# Autodesk Inventor assembly: blue wheel
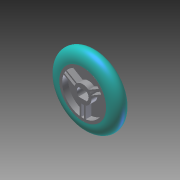
[picture p0: Inventor's stored thumbnail of the model, 180x180]
Saved by Autodesk Inventor 2012 (Build 160160000, 160)
## iProperties
Created: 2013-10-11
Part Number: blue wheel
Document SubType Name: Assembly
Designer: Bryce
Author: Bryce
## Documents named in this file (3)
- C:\Users\Bryce\Dropbox\Inventor Design Project Files\Independent Swerves\Inventor 2012\blue wheel.iam
- C:\Users\Bryce\Dropbox\Inventor Design Project Files\Independent Swerves\Inventor 2012\blue wheel hub.ipt
- C:\Users\Bryce\Dropbox\Inventor Design Project Files\Independent Swerves\Inventor 2012\blue wheel tread.ipt
## Components (2 placed, 2 different names)
1. blue wheel hub:1 — Mate:1, Flush:1
2. blue wheel tread:1 — Mate:1, Flush:1
## Relationships (2: Mate 1, Flush 1)
- Mate:1: blue wheel hub:1 ↔ blue wheel tread:1
- Flush:1: blue wheel hub:1 ↔ blue wheel tread:1
